# Autodesk Inventor assembly: Brodyv2
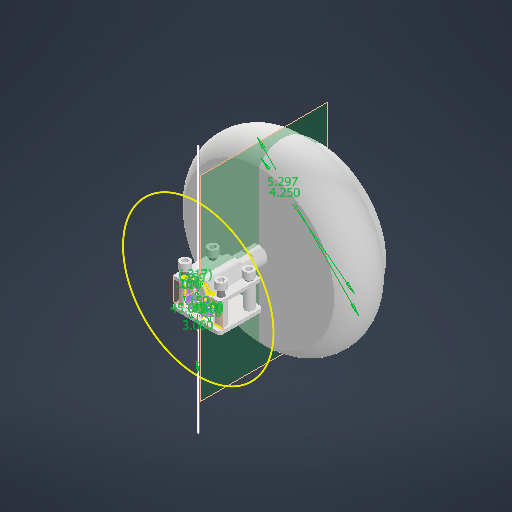
[picture p0: Inventor's stored thumbnail of the model, 512x512]
Saved by Autodesk Inventor 2027 (Build 310192000, 192)
## iProperties
Created: 2026-07-06
Part Number: Brodyv2
Document SubType Name: Assembly
Designer: belcz
Author: belcz
## Documents named in this file (6)
- C:\BrodyProject\Brodyv2.iam
- C:\BrodyProject\Wheel.ipt
- C:\BrodyProject\Wheel Bracket.ipt
- C:\BrodyProject\WheelBracketScrew.ipt
- C:\BrodyProject\WheelBracketConnector.ipt
- C:\BrodyProject\FastenerForLegFrame.ipt
## Components (8 placed, 5 different names)
1. Wheel:1 — Flush:1, Flush:2, Slider:1, Mate:1
2. WheelBracketScrew:1 — Mate:3
3. WheelBracketScrew:2 — Mate:4
4. WheelBracketScrew:3 — Mate:5
5. WheelBracketScrew:4 — Mate:2
6. WheelBracketConnector:1
7. FastenerForLegFrame:1 — Flush:2
8. Wheel Bracket:2 — Slider:1, Mate:1, Mate:2, Mate:3, Mate:4, Mate:5
## Relationships (8: Mate 5, Flush 2, TranslationJoint 1)
- Flush:1 (203.2 mm): Wheel:1
- Flush:2: Wheel:1 ↔ FastenerForLegFrame:1
- Slider:1 [TranslationJoint]: Wheel:1 ↔ Wheel Bracket:2
- Mate:1: Wheel:1 ↔ Wheel Bracket:2
- Mate:2: WheelBracketScrew:4 ↔ Wheel Bracket:2
- Mate:3: WheelBracketScrew:1 ↔ Wheel Bracket:2
- Mate:4: WheelBracketScrew:2 ↔ Wheel Bracket:2
- Mate:5: WheelBracketScrew:3 ↔ Wheel Bracket:2
